# Autodesk Inventor assembly: Top Plate
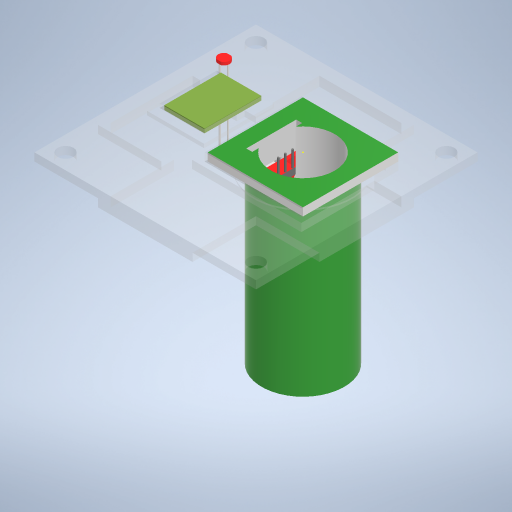
[picture p0: Inventor's stored thumbnail of the model, 512x512]
Saved by Autodesk Inventor 2023 (Build 270158000, 158)
## iProperties
Created: 2023-10-11
Part Number: Top Plate
Document SubType Name: Assembly
Designer: Gage
Author: Gage
## Documents named in this file (5)
- C:\Users\Gage\OneDrive\Desktop\Autodesk Inventor\207\Top Plate.iam
- C:\Users\Gage\OneDrive\Desktop\Autodesk Inventor\207\FinalBoxTop.ipt
- C:\Users\Gage\OneDrive\Desktop\Autodesk Inventor\207\Water Collection Sytem.iam
- C:\Users\Gage\OneDrive\Desktop\Autodesk Inventor\207\PhotoResistor.ipt
- C:\Users\Gage\OneDrive\Desktop\Autodesk Inventor\207\sensor.ipt
## Components (4 placed, 4 different names)
1. FinalBoxTop:1 — Mate:1, Mate:2, Mate:3, Mate:4, Mate:5, Mate:6, Mate:7
2. Water Collection Sytem:1 [sub-assembly] — Mate:3, Mate:4
3. PhotoResistor:1 — Mate:1, Mate:2
4. sensor:1 — Mate:5, Mate:6, Mate:7
## Relationships (7: Mate 7)
- Mate:1: FinalBoxTop:1 ↔ PhotoResistor:1
- Mate:2: FinalBoxTop:1 ↔ PhotoResistor:1
- Mate:3: FinalBoxTop:1 ↔ Water Collection Sytem:1
- Mate:4: FinalBoxTop:1 ↔ Water Collection Sytem:1
- Mate:5: FinalBoxTop:1 ↔ sensor:1
- Mate:6: FinalBoxTop:1 ↔ sensor:1
- Mate:7: FinalBoxTop:1 ↔ sensor:1
